# Autodesk Inventor assembly: INDX_000_Main
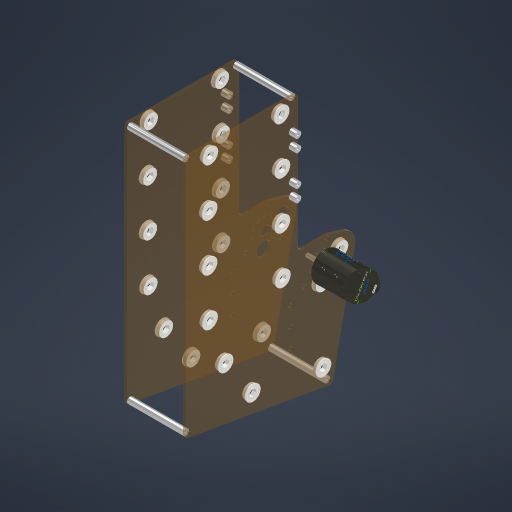
[picture p0: Inventor's stored thumbnail of the model, 512x512]
Saved by Autodesk Inventor 2024.2 (Build 282272000, 272)
## iProperties
Created: 2024-08-08
Part Number: INDX_000_Main
Document SubType Name: Assembly
Designer: Oscar
Author: Oscar
## Documents named in this file (6)
- C:\Users\bobsb\OneDrive\Documents\GitHub\1622-2024-Summer-CAD-A-Thon\Index\INDX_000_Main.iam
- C:\Users\bobsb\OneDrive\Documents\GitHub\1622-2024-Summer-CAD-A-Thon\Index\INDX_001_Plate.ipt
- C:\Users\bobsb\OneDrive\Documents\GitHub\1622-2024-Summer-CAD-A-Thon\Index\INDX_002_Standoff.ipt
- C:\Users\bobsb\OneDrive\Documents\GitHub\1622-2024-Summer-CAD-A-Thon\COTS Library\Motion\Bearings\COTS_WCP-0783_1.125ODHexBearing.ipt
- C:\Users\bobsb\OneDrive\Documents\GitHub\1622-2024-Summer-CAD-A-Thon\COTS Library\Motors\COTS_WCP_Full_Kraken.iam
- C:\Users\bobsb\OneDrive\Documents\GitHub\1622-2024-Summer-CAD-A-Thon\Index\INDX_003_OuterStandoff.ipt
## Components (39 placed, 5 different names)
1. INDX_001_Plate:1 — Mate:1, Mate:2, Mate:4, Mate:7, Mate:8, Mate:11, Mate:32, Mate:33, Mate:34, Mate:35, Mate:36, Mate:37, Mate:38, Mate:39, Mate:40, Mate:41, Mate:42, Mate:43, Mate:44, Mate:45, Mate:46, Mate:47, Mate:48, Mate:49, Mate:50, Mate:51, Mate:52, Mate:53, Mate:71, Mate:72, Mate:73, Mate:74, Mate:75, Mate:76, Mate:77, Mate:78
2. INDX_001_Plate:2 — Mate:1, Mate:2, Mate:3, Mate:5, Mate:6, Mate:9, Mate:10, Mate:12, Mate:13, Mate:14, Mate:15, Mate:16, Mate:17, Mate:18, Mate:19, Mate:20, Mate:21, Mate:22, Mate:23, Mate:24, Mate:25, Mate:26, Mate:27, Mate:28, Mate:29, Mate:30, Mate:31, Mate:54, Mate:55, Mate:56, Mate:57, Mate:58, Mate:59, Mate:60, Mate:61, Mate:62, Mate:63, Mate:64, Mate:65, Mate:66, Mate:67, Mate:68, Mate:69, Mate:70
3. INDX_002_Standoff:1 — Mate:8, Mate:9
4. INDX_002_Standoff:2 — Mate:6, Mate:7
5. INDX_002_Standoff:3 — Mate:10, Mate:11
6. INDX_002_Standoff:4 — Mate:3, Mate:4, Mate:5
7. COTS_WCP-0783_1.125ODHexBearing:1 — Mate:18, Mate:19
8. COTS_WCP-0783_1.125ODHexBearing:2 — Mate:16, Mate:17
9. COTS_WCP-0783_1.125ODHexBearing:3 — Mate:20, Mate:21
10. COTS_WCP-0783_1.125ODHexBearing:4 — Mate:22, Mate:23
11. COTS_WCP-0783_1.125ODHexBearing:5 — Mate:13, Mate:14
12. COTS_WCP-0783_1.125ODHexBearing:6 — Mate:12, Mate:15
13. COTS_WCP-0783_1.125ODHexBearing:7 — Mate:24, Mate:25
14. COTS_WCP-0783_1.125ODHexBearing:8 — Mate:26, Mate:27
15. COTS_WCP-0783_1.125ODHexBearing:9 — Mate:30, Mate:31
16. COTS_WCP-0783_1.125ODHexBearing:10 — Mate:28, Mate:29
17. COTS_WCP-0783_1.125ODHexBearing:11 — Mate:34, Mate:35
18. COTS_WCP-0783_1.125ODHexBearing:12 — Mate:32, Mate:33
19. COTS_WCP-0783_1.125ODHexBearing:13 — Mate:36, Mate:37
20. COTS_WCP-0783_1.125ODHexBearing:14 — Mate:42, Mate:43
21. COTS_WCP-0783_1.125ODHexBearing:15 — Mate:40, Mate:41
22. COTS_WCP-0783_1.125ODHexBearing:16 — Mate:38, Mate:39
23. COTS_WCP-0783_1.125ODHexBearing:17 — Mate:44, Mate:45
24. COTS_WCP-0783_1.125ODHexBearing:18 — Mate:46, Mate:47
25. COTS_WCP-0783_1.125ODHexBearing:19 — Mate:52, Mate:53
26. COTS_WCP-0783_1.125ODHexBearing:20 — Mate:48, Mate:49
27. COTS_WCP-0783_1.125ODHexBearing:21 — Mate:50, Mate:51
28. COTS_WCP_Full_Kraken:1 [sub-assembly] — Mate:54, Mate:55, Mate:56
29. COTS_WCP-0783_1.125ODHexBearing:22 — Mate:59, Mate:60
30. COTS_WCP-0783_1.125ODHexBearing:23 — Mate:57, Mate:58
31. COTS_WCP-0783_1.125ODHexBearing:24 — Mate:61, Mate:62
32. INDX_003_OuterStandoff:1 — Mate:72, Mate:75
33. INDX_003_OuterStandoff:2 — Mate:73, Mate:77
34. INDX_003_OuterStandoff:3 — Mate:63, Mate:68
35. INDX_003_OuterStandoff:4 — Mate:64, Mate:69
36. INDX_003_OuterStandoff:5 — Mate:65, Mate:70
37. INDX_003_OuterStandoff:6 — Mate:66, Mate:67
38. INDX_003_OuterStandoff:7 — Mate:71, Mate:76
39. INDX_003_OuterStandoff:8 — Mate:74, Mate:78
## Relationships (78: Mate 78)
- Mate:1: INDX_001_Plate:1 ↔ INDX_001_Plate:2
- Mate:2: INDX_001_Plate:1 ↔ INDX_001_Plate:2
- Mate:3: INDX_001_Plate:2 ↔ INDX_002_Standoff:4
- Mate:4: INDX_001_Plate:1 ↔ INDX_002_Standoff:4
- Mate:5: INDX_001_Plate:2 ↔ INDX_002_Standoff:4
- Mate:6: INDX_001_Plate:2 ↔ INDX_002_Standoff:2
- Mate:7: INDX_001_Plate:1 ↔ INDX_002_Standoff:2
- Mate:8: INDX_001_Plate:1 ↔ INDX_002_Standoff:1
- Mate:9: INDX_001_Plate:2 ↔ INDX_002_Standoff:1
- Mate:10: INDX_001_Plate:2 ↔ INDX_002_Standoff:3
- Mate:11: INDX_001_Plate:1 ↔ INDX_002_Standoff:3
- Mate:12: INDX_001_Plate:2 ↔ COTS_WCP-0783_1.125ODHexBearing:6
- Mate:13: INDX_001_Plate:2 ↔ COTS_WCP-0783_1.125ODHexBearing:5
- Mate:14: INDX_001_Plate:2 ↔ COTS_WCP-0783_1.125ODHexBearing:5
- Mate:15: INDX_001_Plate:2 ↔ COTS_WCP-0783_1.125ODHexBearing:6
- Mate:16: INDX_001_Plate:2 ↔ COTS_WCP-0783_1.125ODHexBearing:2
- Mate:17: INDX_001_Plate:2 ↔ COTS_WCP-0783_1.125ODHexBearing:2
- Mate:18: INDX_001_Plate:2 ↔ COTS_WCP-0783_1.125ODHexBearing:1
- Mate:19: INDX_001_Plate:2 ↔ COTS_WCP-0783_1.125ODHexBearing:1
- Mate:20: INDX_001_Plate:2 ↔ COTS_WCP-0783_1.125ODHexBearing:3
- Mate:21: INDX_001_Plate:2 ↔ COTS_WCP-0783_1.125ODHexBearing:3
- Mate:22: INDX_001_Plate:2 ↔ COTS_WCP-0783_1.125ODHexBearing:4
- Mate:23: INDX_001_Plate:2 ↔ COTS_WCP-0783_1.125ODHexBearing:4
- Mate:24: INDX_001_Plate:2 ↔ COTS_WCP-0783_1.125ODHexBearing:7
- Mate:25: INDX_001_Plate:2 ↔ COTS_WCP-0783_1.125ODHexBearing:7
- Mate:26: INDX_001_Plate:2 ↔ COTS_WCP-0783_1.125ODHexBearing:8
- Mate:27: INDX_001_Plate:2 ↔ COTS_WCP-0783_1.125ODHexBearing:8
- Mate:28: INDX_001_Plate:2 ↔ COTS_WCP-0783_1.125ODHexBearing:10
- Mate:29: INDX_001_Plate:2 ↔ COTS_WCP-0783_1.125ODHexBearing:10
- Mate:30: INDX_001_Plate:2 ↔ COTS_WCP-0783_1.125ODHexBearing:9
- Mate:31: INDX_001_Plate:2 ↔ COTS_WCP-0783_1.125ODHexBearing:9
- Mate:32: INDX_001_Plate:1 ↔ COTS_WCP-0783_1.125ODHexBearing:12
- Mate:33: INDX_001_Plate:1 ↔ COTS_WCP-0783_1.125ODHexBearing:12
- Mate:34: INDX_001_Plate:1 ↔ COTS_WCP-0783_1.125ODHexBearing:11
- Mate:35: INDX_001_Plate:1 ↔ COTS_WCP-0783_1.125ODHexBearing:11
- Mate:36: INDX_001_Plate:1 ↔ COTS_WCP-0783_1.125ODHexBearing:13
- Mate:37: INDX_001_Plate:1 ↔ COTS_WCP-0783_1.125ODHexBearing:13
- Mate:38: INDX_001_Plate:1 ↔ COTS_WCP-0783_1.125ODHexBearing:16
- Mate:39: INDX_001_Plate:1 ↔ COTS_WCP-0783_1.125ODHexBearing:16
- Mate:40: INDX_001_Plate:1 ↔ COTS_WCP-0783_1.125ODHexBearing:15
- Mate:41: INDX_001_Plate:1 ↔ COTS_WCP-0783_1.125ODHexBearing:15
- Mate:42: INDX_001_Plate:1 ↔ COTS_WCP-0783_1.125ODHexBearing:14
- Mate:43: INDX_001_Plate:1 ↔ COTS_WCP-0783_1.125ODHexBearing:14
- Mate:44: INDX_001_Plate:1 ↔ COTS_WCP-0783_1.125ODHexBearing:17
- Mate:45: INDX_001_Plate:1 ↔ COTS_WCP-0783_1.125ODHexBearing:17
- Mate:46: INDX_001_Plate:1 ↔ COTS_WCP-0783_1.125ODHexBearing:18
- Mate:47: INDX_001_Plate:1 ↔ COTS_WCP-0783_1.125ODHexBearing:18
- Mate:48: INDX_001_Plate:1 ↔ COTS_WCP-0783_1.125ODHexBearing:20
- Mate:49: INDX_001_Plate:1 ↔ COTS_WCP-0783_1.125ODHexBearing:20
- Mate:50: INDX_001_Plate:1 ↔ COTS_WCP-0783_1.125ODHexBearing:21
- Mate:51: INDX_001_Plate:1 ↔ COTS_WCP-0783_1.125ODHexBearing:21
- Mate:52: INDX_001_Plate:1 ↔ COTS_WCP-0783_1.125ODHexBearing:19
- Mate:53: INDX_001_Plate:1 ↔ COTS_WCP-0783_1.125ODHexBearing:19
- Mate:54: INDX_001_Plate:2 ↔ COTS_WCP_Full_Kraken:1
- Mate:55: INDX_001_Plate:2 ↔ COTS_WCP_Full_Kraken:1
- Mate:56: INDX_001_Plate:2 ↔ COTS_WCP_Full_Kraken:1
- Mate:57: INDX_001_Plate:2 ↔ COTS_WCP-0783_1.125ODHexBearing:23
- Mate:58: INDX_001_Plate:2 ↔ COTS_WCP-0783_1.125ODHexBearing:23
- Mate:59: INDX_001_Plate:2 ↔ COTS_WCP-0783_1.125ODHexBearing:22
- Mate:60: INDX_001_Plate:2 ↔ COTS_WCP-0783_1.125ODHexBearing:22
- Mate:61: INDX_001_Plate:2 ↔ COTS_WCP-0783_1.125ODHexBearing:24
- Mate:62: INDX_001_Plate:2 ↔ COTS_WCP-0783_1.125ODHexBearing:24
- Mate:63: INDX_001_Plate:2 ↔ INDX_003_OuterStandoff:3
- Mate:64: INDX_001_Plate:2 ↔ INDX_003_OuterStandoff:4
- Mate:65: INDX_001_Plate:2 ↔ INDX_003_OuterStandoff:5
- Mate:66: INDX_001_Plate:2 ↔ INDX_003_OuterStandoff:6
- Mate:67: INDX_001_Plate:2 ↔ INDX_003_OuterStandoff:6
- Mate:68: INDX_001_Plate:2 ↔ INDX_003_OuterStandoff:3
- Mate:69: INDX_001_Plate:2 ↔ INDX_003_OuterStandoff:4
- Mate:70: INDX_001_Plate:2 ↔ INDX_003_OuterStandoff:5
- Mate:71: INDX_001_Plate:1 ↔ INDX_003_OuterStandoff:7
- Mate:72: INDX_001_Plate:1 ↔ INDX_003_OuterStandoff:1
- Mate:73: INDX_001_Plate:1 ↔ INDX_003_OuterStandoff:2
- Mate:74: INDX_001_Plate:1 ↔ INDX_003_OuterStandoff:8
- Mate:75: INDX_001_Plate:1 ↔ INDX_003_OuterStandoff:1
- Mate:76: INDX_001_Plate:1 ↔ INDX_003_OuterStandoff:7
- Mate:77: INDX_001_Plate:1 ↔ INDX_003_OuterStandoff:2
- Mate:78: INDX_001_Plate:1 ↔ INDX_003_OuterStandoff:8
